# Autodesk Inventor assembly: PCB
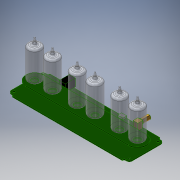
[picture p0: Inventor's stored thumbnail of the model, 180x180]
Saved by Autodesk Inventor 2017 (Build 210142000, 142)
## iProperties
Created: 2017-04-18
Part Number: PCB
Document SubType Name: Assembly
Designer: jeffkub
Author: jeffkub
## Documents named in this file (4)
- C:\Projects\nixie-clock\mechanical\PCB.iam
- C:\Projects\nixie-clock\mechanical\MainPCB.ipt
- C:\Projects\nixie-clock\mechanical\TubePCB.ipt
- C:\Projects\nixie-clock\mechanical\IN-14.ipt
## Components (8 placed, 3 different names)
1. MainPCB:1 — Flush:1, Flush:2, Flush:3, Mate:1
2. TubePCB:1 — Mate:1, Flush:4, Flush:5, Mate:2, Mate:3, Mate:4, Mate:5, Mate:6, Mate:7, Mate:8, Mate:9, Mate:10, Mate:11, Mate:12, Mate:13
3. IN-14:1 — Mate:2, Mate:8
4. IN-14:2 — Mate:3, Mate:9
5. IN-14:3 — Mate:4, Mate:10
6. IN-14:4 — Mate:5, Mate:11
7. IN-14:5 — Mate:6, Mate:12
8. IN-14:6 — Mate:7, Mate:13
## Relationships (18: Mate 13, Flush 5)
- Flush:1: MainPCB:1
- Flush:2: MainPCB:1
- Flush:3: MainPCB:1
- Mate:1 (7.1 mm): MainPCB:1 ↔ TubePCB:1
- Flush:4: TubePCB:1
- Flush:5: TubePCB:1
- Mate:2: TubePCB:1 ↔ IN-14:1
- Mate:3: TubePCB:1 ↔ IN-14:2
- Mate:4: TubePCB:1 ↔ IN-14:3
- Mate:5: TubePCB:1 ↔ IN-14:4
- Mate:6: TubePCB:1 ↔ IN-14:5
- Mate:7: TubePCB:1 ↔ IN-14:6
- Mate:8: TubePCB:1 ↔ IN-14:1
- Mate:9: TubePCB:1 ↔ IN-14:2
- Mate:10: TubePCB:1 ↔ IN-14:3
- Mate:11: TubePCB:1 ↔ IN-14:4
- Mate:12: TubePCB:1 ↔ IN-14:5
- Mate:13: TubePCB:1 ↔ IN-14:6
